# Autodesk Inventor assembly: TZS 1230 inner elbow
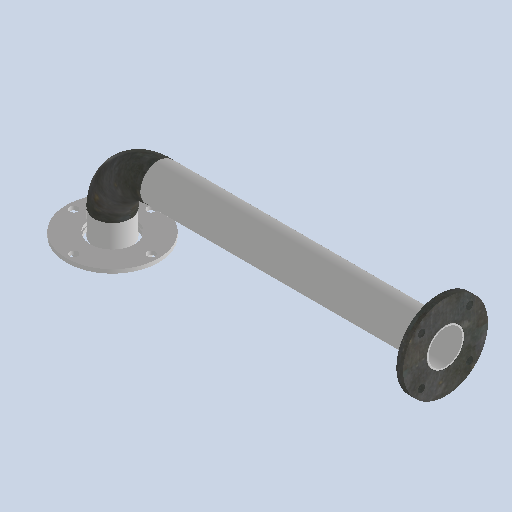
[picture p0: Inventor's stored thumbnail of the model, 512x512]
Saved by Autodesk Inventor 2025 (Build 290162010, 162A)
## iProperties
Created: 2025-07-04
Part Number: TZS 1230 inner elbow
Document SubType Name: Assembly
Designer: user
Author: user
## Documents named in this file (7)
- C:\Users\pokla\Documents\Inventor\TZS-Tazovskiy\Фильтр D1200\TZS 1230 inner elbow.iam
- C:\Users\pokla\Documents\Inventor\TZS-Tazovskiy\Фильтр D1200\TZS 1233 FDS tube 3.ipt
- C:\Users\pokla\Documents\Inventor\TZS-Tazovskiy\Фильтр D1200\TZS 1231 FDS flange DN90.ipt
- C:\Users\pokla\Documents\Inventor\TZS-Tazovskiy\Фильтр D1200\TZS 1232 FDS free flange DN90.ipt
- C:\Users\pokla\Documents\Inventor\TZS-Tazovskiy\Фильтр D1200\TZS 1234 FDS tube 4.ipt
- C:\Users\pokla\Documents\Inventor\Content Center Files\R2025\en-US\JIS B 2220 SOP - 10K(2)\JIS B 2220 Slip-On Welding Thin Plate Type Flange SOP - 10K 65.ipt
- C:\Users\pokla\Documents\Inventor\Content Center Files\R2025\en-US\JIS B 2312 90 (2)\JIS B 2312 90 Deg Long Elbow Steel 65A x Sch 40.ipt
## Components (6 placed, 6 different names)
1. JIS B 2312 90 Deg Long Elbow Steel 100A x Sch 40.ipt:1
2. TZS 1233 FDS tube 3.ipt:1 — Rigid:7
3. TZS 1234 FDS tube 4.ipt:1
4. TZS 1231 FDS flange DN90.ipt:1
5. TZS 1232 FDS free flange DN90.ipt:1
6. DIN 2576 Slip-On Flange for Welding Series 1 (ISO) - PN 10 80 x 88.9.ipt:1 — Rigid:7
## Relationships (5: WeldJoint 5)
- [WeldJoint]: JIS B 2312 90 Deg Long Elbow Steel 100A x Sch 40.ipt:1 ↔ TZS 1233 FDS tube 3.ipt:1
- [WeldJoint]: JIS B 2312 90 Deg Long Elbow Steel 100A x Sch 40.ipt:1 ↔ TZS 1234 FDS tube 4.ipt:1
- [WeldJoint]: TZS 1234 FDS tube 4.ipt:1 ↔ TZS 1232 FDS free flange DN90.ipt:1
- [WeldJoint]: TZS 1231 FDS flange DN90.ipt:1 ↔ TZS 1232 FDS free flange DN90.ipt:1
- Rigid:7 [WeldJoint]: TZS 1233 FDS tube 3.ipt:1 ↔ DIN 2576 Slip-On Flange for Welding Series 1 (ISO) - PN 10 80 x 88.9.ipt:1
